(part 1 of 2)
# Autodesk Inventor assembly: Drive Roller Assembly 3 (Lexan)
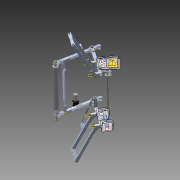
[picture p0: Inventor's stored thumbnail of the model, 180x180]
Saved by Autodesk Inventor 2014 (Build 180170000, 170)
## iProperties
Created: 2014-01-12
Part Number: Drive Roller Assembly 3 (Lexan)
Document SubType Name: Assembly
Designer: Michael
Mass: 8436.07 g
Surface Area: 19089.5 cm^2
Volume: 2323.39 cm^3
Density: 3.63094 g/cm^3
Author: Michael
## Documents named in this file (43)
- C:\Users\Michael\Documents\GitHub\2014buildCAD\Duluth Collector\Drive Roller Assembly 3 (Lexan).iam
- C:\Users\Michael\Documents\GitHub\2014buildCAD\Collector\Roller End Cap Drive (3-D Printed).ipt
- C:\Users\Michael\Documents\GitHub\2014buildCAD\Collector\VersaPlanetary (Fixed).iam
- C:\Users\Michael\Documents\GitHub\2014buildCAD\New Collector\Polycarbonate Roller 2 OD 1-16 Thick (8585K64).ipt
- C:\Users\Michael\Documents\GitHub\2014buildCAD\New Collector\Hex Bearing 1-2 in (FR8ZZ-Hex, am-0279).ipt
- C:\Users\Michael\Documents\GitHub\2014buildCAD\New Collector\Hex Shaft Collar 1-2 in (7552K500).ipt
- C:\Users\Michael\Documents\GitHub\2014buildCAD\New Collector\Roller End Cap Drive (3-D Printed).ipt
- C:\Users\Michael\Documents\GitHub\2014buildCAD\New Collector\Vex Pro End Bearing Mount.ipt
- C:\Users\Michael\Documents\GitHub\2014buildCAD\New Collector\Vex Pro 1x1 rectangular tubing 14 in length.ipt
- C:\Users\Michael\Documents\GitHub\2014buildCAD\New Collector\Hex Shaft Aluminum 1-2 in (am-2291).ipt
- C:\Users\Michael\Documents\GitHub\2014buildCAD\New Collector\Timing Pulley (HTD 5mm) - 18T 9mm Double Flange, 1-2 in Hex (VexPro).ipt
- C:\Users\Michael\Documents\GitHub\2014buildCAD\New Collector\Vex Pro 90 degree gusset.ipt
- C:\Users\Michael\Documents\GitHub\2014buildCAD\New Collector\Vex Pro 1x1 rectangular tubing 2 in length.ipt
- C:\Users\Michael\Documents\GitHub\2014buildCAD\New Collector\Hex Shaft 3-8 in (am-0855).ipt
- C:\Users\Michael\Documents\GitHub\2014buildCAD\New Collector\Hex Shaft Collar 3-8 in (7552K300).ipt
- C:\Users\Michael\Documents\GitHub\2014buildCAD\New Collector\Hex Shaft 1-2 in (am-0856).ipt
- C:\Users\Michael\Documents\GitHub\2014buildCAD\New Collector\Vex Pro 1x1 rectangular tubing 4 in length.ipt
- C:\Users\Michael\Documents\GitHub\2014buildCAD\New Collector\Pneumatic Piston Front Flange (Lt Custom).ipt
- C:\Users\Michael\Documents\GitHub\2014buildCAD\New Collector\Pneumatic Piston Front Flange (Rt Custom).ipt
- C:\Users\Michael\Documents\GitHub\2014buildCAD\New Collector\Pneumatic Piston Back Flange (Rt Custom).ipt
- C:\Users\Michael\Documents\GitHub\2014buildCAD\New Collector\Vex Pro 1x1 rectangular tubing 14 in length (roller).ipt
- C:\Users\Michael\Documents\GitHub\2014buildCAD\New Collector\Pneumatic Piston Back Flange (Right Custom).ipt
- C:\Users\Michael\Documents\GitHub\2014buildCAD\New Collector\Hex Shaft 1-2 in 5 in long (am-0856).ipt
- C:\Users\Michael\Documents\GitHub\2014buildCAD\New Collector\Vex Pro End Bearing Mount (Bolt).ipt
- C:\Users\Michael\Documents\GitHub\2014buildCAD\New Collector\Bracket.ipt
- C:\Users\Michael\Documents\GitHub\2014buildCAD\New Collector\Shaft Collar 3-16 in ID (6435K510).ipt
- C:\Users\Michael\Documents\GitHub\2014buildCAD\New Collector\Standoff #8 (91125A459).ipt
- C:\Users\Michael\Documents\GitHub\2014buildCAD\New Collector\Vex Pro 1x1 rectangular tubing 21.375 in length.ipt
- C:\Users\Michael\Documents\GitHub\2014buildCAD\New Collector\Roller Crossbar Gusset (Custom).ipt
- C:\Users\Michael\Documents\GitHub\2014buildCAD\New Collector\Vex Pro 1x1 rectangular tubing 2 in length (Flange Support).ipt
- C:\Users\Michael\Documents\GitHub\2014buildCAD\New Collector\Vex Pro 90 degree gusset (1-8 in).ipt
- C:\Users\Michael\Documents\GitHub\2014buildCAD\New Collector\Timing Pulley (HTD 5mm) - 18T 15mm 1-2 in Hex.ipt
- C:\Users\Michael\Documents\GitHub\2014buildCAD\New Collector\Hex Spacer.ipt
- C:\Users\Michael\Documents\GitHub\2014buildCAD\New Collector\Side Mount Custom.ipt
- C:\Users\Michael\Documents\GitHub\2014buildCAD\New Collector\Clamp Piston ( 1 in stroke twice, 9-16 bore).iam
- C:\Users\Michael\Documents\GitHub\2014buildCAD\New Collector\Hex Spacer 1-2 .ipt
- C:\Users\Michael\Documents\GitHub\2014buildCAD\New Collector\Lexan flexible Arm Mount.ipt
- C:\Users\Michael\Documents\GitHub\2014buildCAD\New Collector\Hex Shaft Connector (Lexan).ipt
- C:\Users\Michael\Documents\GitHub\2014buildCAD\New Collector\Clamp with Piston Assembly (new).iam
- C:\Users\Michael\Documents\GitHub\2014buildCAD\Duluth Collector\Vex Pro T gusset - OUT OF STOCK 1192014.ipt
- C:\Users\Michael\Documents\GitHub\2014buildCAD\Duluth Collector\Vex Pro 1x1 rectangular tubing 2 in length (no hex).ipt
- C:\Users\Michael\Documents\GitHub\2014buildCAD\Duluth Collector\Torsion Spring 10 in-lb (9271K621).ipt
- C:\Users\Michael\Documents\GitHub\2014buildCAD\Duluth Collector\Bearing Mount Spacer 1-8 in.ipt
## Components (143 placed, 41 different names)
1. Roller End Cap Drive (3-D Printed):2 — Mate:154, Mate:155, Mate:1112, Flush:30, Mate:1114, Mate:1115
2. VersaPlanetary (Fixed):1 [sub-assembly] — Mate:990, Mate:991, Mate:992, Mate:1076, Mate:1077, Mate:1079, Mate:1080, Mate:1082, Mate:1083
3. Hex Bearing 1-2 in (FR8ZZ-Hex, am-0279):3 — Mate:128, Mate:129, Mate:134, Mate:1113
4. Roller End Cap Drive (3-D Printed):5 — Mate:1108, Mate:1109, Mate:1110
5. Hex Shaft Aluminum 1-2 in (am-2291):1 — Mate:132, Mate:134, Mate:154, Mate:155, Mate:172, Mate:173, Mate:179, Mate:180, Mate:467, Mate:468, Mate:1065, Mate:1066, Mate:1068, Mate:1069, Mate:1072, Mate:1073, Flush:30
6. Vex Pro End Bearing Mount:4 — Mate:130, Mate:131, Mate:621, Mate:798, Mate:799, Mate:873
7. Vex Pro End Bearing Mount:5 — Mate:128, Mate:129, Mate:624, Mate:800, Mate:801, Mate:866, Mate:867, Mate:868, Mate:869, Mate:870, Mate:871, Mate:872
8. Hex Bearing 1-2 in (FR8ZZ-Hex, am-0279):4 — Mate:130, Mate:131, Mate:132, Mate:1067
9. Hex Bearing 1-2 in (FR8ZZ-Hex, am-0279):5 — Mate:178, Mate:758, Mate:759
10. Vex Pro End Bearing Mount:7 — Mate:631, Mate:804, Mate:805
11. Vex Pro End Bearing Mount:8 — Mate:629, Mate:802, Mate:803, Mate:874, Mate:875, Mate:876, Mate:877, Mate:878, Mate:879, Mate:880, Mate:881
12. Hex Bearing 1-2 in (FR8ZZ-Hex, am-0279):6 — Mate:172, Mate:173, Mate:470, Mate:471, Mate:1111
13. Hex Shaft Collar 1-2 in (7552K500):16 — Mate:178, Mate:179, Mate:180, Flush:13
14. Vex Pro 1x1 rectangular tubing 14 in length:5 — Mate:203, Mate:210, Mate:211, Mate:221, Mate:222, Mate:223, Flush:20, Mate:940, Mate:942, Mate:979, Mate:981, Flush:27, Mate:1084, Mate:1085, Mate:1140, Mate:1141, Mate:1146, Mate:1147, Mate:1148, Mate:1184, Mate:1185, Mate:1186, Mate:1190, Mate:1191, Mate:1192, Mate:1218, Mate:1219, Mate:1220, Mate:1224, Mate:1225, Mate:1226, Mate:1246, Mate:1247, Mate:1248, Mate:1250, Mate:1251, Mate:1252
15. Vex Pro 1x1 rectangular tubing 14 in length:6 — Mate:258, Mate:259, Mate:260, Mate:263, Mate:320, Mate:321, Flush:20, Mate:935, Mate:936, Mate:938, Mate:977, Flush:26, Mate:1092, Mate:1117, Mate:1129, Mate:1130, Mate:1131, Mate:1132, Mate:1230, Mate:1231, Mate:1232, Mate:1236, Mate:1237, Mate:1238, Mate:1254, Mate:1255, Mate:1256, Mate:1260, Mate:1261, Mate:1262
16. Vex Pro 90 degree gusset:8 — Mate:203, Mate:210, Mate:211, Mate:212, Mate:213, Mate:214
17. Vex Pro 1x1 rectangular tubing 2 in length:1 — Mate:212, Mate:213, Mate:214, Flush:25, Mate:941, Mate:961, Mate:962, Mate:964, Mate:965, Flush:37
18. Vex Pro 90 degree gusset:10 — Mate:221, Mate:222, Mate:223
19. Vex Pro 1x1 rectangular tubing 2 in length:2 — Mate:224, Mate:225, Mate:967, Mate:968, Mate:970, Mate:971, Mate:1086, Flush:38
20. Hex Shaft 3-8 in (am-0855):1 — Mate:224, Mate:225, Mate:228, Mate:229, Mate:231, Mate:232, Mate:919, Mate:920, Mate:922, Mate:923, Mate:963, Mate:966, Mate:969, Mate:972, Flush:32, Flush:33
21. Hex Shaft Collar 3-8 in (7552K300):1 — Mate:228, Mate:229, Mate:1163, Mate:1167, Mate:1242, Mate:1243, Flush:41
22. Hex Shaft Collar 3-8 in (7552K300):2 — Mate:231, Mate:232, Mate:1164, Flush:32
23. Vex Pro 90 degree gusset:12 — Mate:263, Mate:320, Mate:321
24. Vex Pro 1x1 rectangular tubing 2 in length:3 — Flush:25, Mate:949, Mate:950, Mate:952, Mate:953, Flush:40
25. Vex Pro 90 degree gusset:13 — Mate:258, Mate:259, Mate:260
26. Vex Pro 1x1 rectangular tubing 2 in length:4 — Mate:955, Mate:956, Mate:958, Mate:959, Mate:1090, Mate:1091
27. Hex Shaft 3-8 in (am-0855):2 — Mate:915, Mate:917, Mate:925, Mate:926, Mate:951, Mate:954, Mate:957, Mate:960, Flush:34
28. Hex Shaft Collar 3-8 in (7552K300):3 — Mate:1170, Mate:1183, Mate:1244, Mate:1245, Flush:42
29. Hex Shaft Collar 3-8 in (7552K300):4 — Mate:1159, Flush:34
30. Hex Shaft Collar 1-2 in (7552K500):18 — Mate:1150
31. Hex Shaft Collar 1-2 in (7552K500):19 — Mate:1149
32. Hex Shaft Collar 1-2 in (7552K500):20 — Mate:706, Mate:707, Mate:945
33. Hex Shaft Collar 1-2 in (7552K500):21 — Mate:704, Mate:705, Flush:22, Mate:1136
34. Hex Shaft Collar 1-2 in (7552K500):22 — Mate:467, Mate:468, Mate:1112, Mate:1113
35. Hex Shaft Aluminum 1-2 in (am-2291):2 — Mate:470, Mate:471, Flush:13, Mate:633, Mate:634, Mate:758, Mate:759, Mate:1108, Mate:1109
36. Vex Pro 1x1 rectangular tubing 4 in length:1 — Mate:683, Mate:684, Mate:685, Mate:1249, Mate:1253, Mate:1258, Mate:1265
37. Vex Pro 1x1 rectangular tubing 4 in length:2 — Mate:694, Mate:699, Mate:700, Mate:1257, Mate:1259, Mate:1263, Mate:1264
38. Hex Bearing 1-2 in (FR8ZZ-Hex, am-0279):7 — Flush:15, Mate:560, Mate:561, Flush:23, Mate:754, Mate:755, Mate:830
39. Hex Shaft 1-2 in (am-0856):4 — Mate:560, Mate:561, Mate:562, Mate:563, Flush:23, Mate:774, Mate:829, Mate:831, Mate:833, Mate:834, Mate:1040, Mate:1043
40. Hex Bearing 1-2 in (FR8ZZ-Hex, am-0279):8 — Flush:15, Mate:746, Mate:747, Mate:774, Mate:832
41. Vex Pro 1x1 rectangular tubing 14 in length (roller):1 — Mate:562, Mate:563, Mate:621, Mate:624, Mate:790, Mate:791, Mate:793, Mate:798, Mate:799, Mate:800, Mate:801, Mate:862, Mate:863, Mate:864, Mate:912, Mate:988, Mate:989, Mate:1038, Mate:1039, Mate:1041, Mate:1042, Flush:26, Mate:1050, Mate:1195, Mate:1196, Mate:1214, Mate:1215, Mate:1216
42. Hex Bearing 1-2 in (FR8ZZ-Hex, am-0279):9 — Flush:19, Mate:752, Mate:753, Mate:854
43. Hex Shaft 1-2 in (am-0856):5 — Flush:19, Mate:775, Mate:836, Mate:843, Mate:852, Mate:853, Mate:1046, Mate:1049
44. Hex Bearing 1-2 in (FR8ZZ-Hex, am-0279):10 — Mate:738, Mate:739, Mate:775, Mate:835
45. Vex Pro 1x1 rectangular tubing 14 in length (roller):2 — Mate:629, Mate:631, Mate:802, Mate:803, Mate:804, Mate:805, Mate:806, Mate:807, Mate:808, Mate:809, Mate:810, Mate:811, Mate:892, Mate:1044, Mate:1045, Mate:1047, Mate:1048, Flush:27, Mate:1197, Mate:1198, Mate:1211, Mate:1212
46. Hex Shaft Collar 1-2 in (7552K500):23 — Mate:633, Mate:634, Mate:1110, Mate:1111
47. Pneumatic Piston Front Flange (Rt Custom):2 — Mate:932, Mate:933, Mate:934, Mate:1155, Mate:1156, Mate:1157
48. Pneumatic Piston Front Flange (Lt Custom):1 — Mate:929, Mate:930, Mate:931, Mate:1160, Mate:1161, Mate:1162
49. Pneumatic Piston Back Flange (Rt Custom):1 — Mate:683, Mate:684, Mate:685, Mate:1028, Mate:1029, Mate:1030
50. Pneumatic Piston Back Flange (Right Custom):1 — Mate:694, Mate:699, Mate:700, Mate:1024, Mate:1025, Mate:1026
51. Hex Shaft 1-2 in 5 in long (am-0856):1 — Mate:704, Mate:705, Mate:706, Mate:707, Flush:22, Mate:714, Mate:715, Mate:946, Mate:947, Mate:1032, Mate:1033, Mate:1133, Mate:1135
52. Hex Shaft Collar 1-2 in (7552K500):24 — Mate:714, Mate:715, Mate:948
53. Vex Pro End Bearing Mount (Bolt):1 — Mate:738, Mate:739, Mate:979, Mate:1221, Mate:1222, Mate:1223
54. Vex Pro End Bearing Mount (Bolt):2 — Mate:752, Mate:753, Mate:981, Mate:1227, Mate:1228, Mate:1229
55. Vex Pro End Bearing Mount (Bolt):3 — Mate:746, Mate:747, Mate:1233, Mate:1234, Mate:1235
56. Vex Pro End Bearing Mount (Bolt):4 — Mate:754, Mate:755, Mate:977, Mate:1239, Mate:1240, Mate:1241
57. Bracket:1 — Mate:790, Mate:791, Mate:793, Mate:860
58. Bracket:2 — Mate:806, Mate:807, Mate:808, Mate:856
59. Bracket:3 — Mate:809, Mate:810, Mate:811, Mate:858
60. Hex Shaft Collar 1-2 in (7552K500):25 — Mate:829, Mate:830, Mate:831
61. Hex Shaft Collar 1-2 in (7552K500):26 — Mate:832, Mate:833, Mate:834
62. Hex Shaft Collar 1-2 in (7552K500):27 — Mate:835, Mate:836, Mate:843
63. Hex Shaft Collar 1-2 in (7552K500):29 — Mate:852, Mate:853, Mate:854
64. Shaft Collar 3-16 in ID (6435K510):1 — Mate:858
65. Shaft Collar 3-16 in ID (6435K510):2 — Mate:856
66. Shaft Collar 3-16 in ID (6435K510):3 — Mate:860
67. Shaft Collar 3-16 in ID (6435K510):4 — Mate:865
68. Bracket:4 — Mate:862, Mate:863, Mate:864, Mate:865
69. Standoff #8 (91125A459):1 — Mate:866, Mate:867
70. Standoff #8 (91125A459):2 — Mate:868, Mate:869
71. Standoff #8 (91125A459):3 — Mate:870, Mate:871
72. Standoff #8 (91125A459):4 — Mate:872, Mate:873
73. Standoff #8 (91125A459):5 — Mate:874, Mate:875
74. Standoff #8 (91125A459):6 — Mate:876, Mate:877
75. Standoff #8 (91125A459):7 — Mate:878, Mate:879
76. Standoff #8 (91125A459):8 — Mate:880, Mate:881
77. Vex Pro 1x1 rectangular tubing 21.375 in length:1 — Mate:894, Mate:1199, Mate:1213
78. Roller Crossbar Gusset (Custom):4 — Mate:892, Mate:894, Mate:1197, Mate:1198, Mate:1199
79. Roller Crossbar Gusset (Custom):5 — Mate:912, Mate:1195, Mate:1196
80. Hex Shaft Collar 3-8 in (7552K300):5 — Mate:915, Mate:917, Mate:1206
81. Hex Shaft Collar 3-8 in (7552K300):6 — Mate:919, Mate:920, Mate:1205
82. Hex Shaft Collar 3-8 in (7552K300):7 — Mate:922, Mate:923, Mate:1166
83. Hex Shaft Collar 3-8 in (7552K300):8 — Mate:925, Mate:926, Mate:1168
84. Vex Pro 1x1 rectangular tubing 2 in length (Flange Support):1 — Mate:929, Mate:930, Mate:931
85. Vex Pro 1x1 rectangular tubing 2 in length (Flange Support):2 — Mate:932, Mate:933, Mate:934
86. Vex Pro 90 degree gusset (1-8 in):1 — Mate:935, Mate:936, Mate:938
87. Vex Pro 90 degree gusset (1-8 in):2 — Mate:940, Mate:941, Mate:942
88. Timing Pulley (HTD 5mm) - 18T 15mm 1-2 in Hex:1 — Mate:945, Mate:946, Mate:947, Mate:948
89. Hex Spacer:1 — Mate:949, Mate:950, Mate:951
90. Hex Spacer:2 — Mate:952, Mate:953, Mate:954
91. Hex Spacer:3 — Mate:955, Mate:956, Mate:957
92. Hex Spacer:4 — Mate:958, Mate:959, Mate:960
93. Hex Spacer:5 — Mate:961, Mate:962, Mate:963
94. Hex Spacer:6 — Mate:964, Mate:965, Mate:966
95. Hex Spacer:7 — Mate:967, Mate:968, Mate:969, Flush:33
96. Hex Spacer:8 — Mate:970, Mate:971, Mate:972
97. Side Mount Custom:1 — Mate:988, Mate:989, Mate:990, Mate:991, Mate:992, Mate:1050
98. Clamp Piston ( 1 in stroke twice, 9-16 bore):1 [sub-assembly] — Mate:1024, Mate:1025, Mate:1026
99. Clamp Piston ( 1 in stroke twice, 9-16 bore):2 [sub-assembly] — Mate:1028, Mate:1029, Mate:1030
100. Hex Shaft Collar 1-2 in (7552K500):30 — Mate:1032, Mate:1033, Mate:1134
101. Hex Spacer 1-2 :1 — Mate:1038, Mate:1039, Mate:1040
102. Hex Spacer 1-2 :2 — Mate:1041, Mate:1042, Mate:1043
103. Hex Spacer 1-2 :3 — Mate:1044, Mate:1045, Mate:1046
104. Hex Spacer 1-2 :4 — Mate:1047, Mate:1048, Mate:1049
105. Hex Shaft Collar 1-2 in (7552K500):31 — Mate:1065, Mate:1066, Mate:1067, Mate:1070
106. Timing Pulley (HTD 5mm) - 18T 9mm Double Flange, 1-2 in Hex (VexPro):5 — Mate:1068, Mate:1069, Mate:1070, Mate:1071
107. Hex Shaft Collar 1-2 in (7552K500):32 — Mate:1071, Mate:1072, Mate:1073, Flush:29
108. Hex Shaft Collar 1-2 in (7552K500):33 — Mate:1081, Mate:1082, Mate:1083
109. Timing Pulley (HTD 5mm) - 18T 9mm Double Flange, 1-2 in Hex (VexPro):6 — Mate:1078, Mate:1079, Mate:1080, Mate:1081
110. Hex Shaft Collar 1-2 in (7552K500):34 — Mate:1076, Flush:29, Mate:1077, Mate:1078
111. Vex Pro 90 degree gusset (1-8 in):3 — Mate:1084, Mate:1085, Mate:1086
112. Vex Pro 90 degree gusset (1-8 in):4 — Mate:1090, Mate:1091, Mate:1092
113. Polycarbonate Roller 2 OD 1-16 Thick (8585K64):1 — Mate:1114, Mate:1115
114. Lexan flexible Arm Mount:1 — Mate:1117, Mate:1126, Mate:1127, Mate:1128, Mate:1129, Mate:1130, Mate:1153
115. Lexan flexible Arm Mount:2 — Mate:1123, Mate:1124, Mate:1125, Mate:1131, Mate:1132, Mate:1153
116. Hex Shaft Connector (Lexan):1 — Mate:1123, Mate:1124, Mate:1125, Mate:1133, Mate:1134
117. Hex Shaft Connector (Lexan):2 — Mate:1126, Mate:1127, Mate:1128, Mate:1135, Mate:1136
118. Lexan flexible Arm Mount:3 — Mate:1140, Mate:1141, Mate:1154
119. Hex Shaft Connector (Lexan):3 — Mate:1150
120. Lexan flexible Arm Mount:4 — Mate:1146, Mate:1147, Mate:1148, Mate:1154
121. Hex Shaft Connector (Lexan):4 — Mate:1149
122. Clamp with Piston Assembly (new):1 [sub-assembly] — Mate:1155, Mate:1156, Mate:1157, Mate:1159, Mate:1168, Mate:1170, Mate:1183, Mate:1206, Mate:1207, Mate:1208
123. Clamp with Piston Assembly (new):2 [sub-assembly] — Mate:1160, Mate:1161, Mate:1162, Mate:1163, Mate:1164, Mate:1166, Mate:1167, Mate:1203, Mate:1204, Mate:1205
124. Vex Pro 1x1 rectangular tubing 4 in length:3 — Mate:1187, Flush:35, Mate:1194
125. Vex Pro T gusset - OUT OF STOCK 1192014:1 — Mate:1184, Mate:1185, Mate:1186, Mate:1187, Flush:35, Mate:1188, Mate:1189, Flush:36
126. Vex Pro 1x1 rectangular tubing 2 in length (no hex):1 — Mate:1188, Mate:1189, Flush:36, Mate:1193
127. Vex Pro T gusset - OUT OF STOCK 1192014:2 — Mate:1190, Mate:1191, Mate:1192, Mate:1193, Mate:1194
128. Torsion Spring 10 in-lb (9271K621):1 — Mate:1203, Flush:37
129. Torsion Spring 10 in-lb (9271K621):2 — Mate:1204, Flush:38
130. Torsion Spring 10 in-lb (9271K621):3 — Mate:1207
131. Torsion Spring 10 in-lb (9271K621):4 — Mate:1208, Flush:40
132. Roller Crossbar Gusset (Custom):6 — Mate:1211, Mate:1212, Mate:1213
133. Roller Crossbar Gusset (Custom):7 — Mate:1214, Mate:1215, Mate:1216
134. Bearing Mount Spacer 1-8 in:1 — Mate:1218, Mate:1219, Mate:1220, Mate:1221, Mate:1222, Mate:1223
135. Bearing Mount Spacer 1-8 in:2 — Mate:1224, Mate:1225, Mate:1226, Mate:1227, Mate:1228, Mate:1229
136. Bearing Mount Spacer 1-8 in:3 — Mate:1230, Mate:1231, Mate:1232, Mate:1233, Mate:1234, Mate:1235
137. Bearing Mount Spacer 1-8 in:5 — Mate:1236, Mate:1237, Mate:1238, Mate:1239, Mate:1240, Mate:1241
138. Hex Shaft 3-8 in (am-0855):3 — Mate:1242, Mate:1243, Flush:41
139. Hex Shaft 3-8 in (am-0855):4 — Mate:1244, Mate:1245, Flush:42
140. Vex Pro T gusset - OUT OF STOCK 1192014:3 — Mate:1246, Mate:1247, Mate:1248, Mate:1249, Mate:1258, Mate:1265
141. Vex Pro T gusset - OUT OF STOCK 1192014:4 — Mate:1250, Mate:1251, Mate:1252, Mate:1253
142. Vex Pro T gusset - OUT OF STOCK 1192014:5 — Mate:1254, Mate:1255, Mate:1256, Mate:1257, Mate:1259
143. Vex Pro T gusset - OUT OF STOCK 1192014:6 — Mate:1260, Mate:1261, Mate:1262, Mate:1263, Mate:1264
## Relationships (400: Mate 378, Flush 22)
- Mate:128: Hex Bearing 1-2 in (FR8ZZ-Hex, am-0279):3 ↔ Vex Pro End Bearing Mount:5
- Mate:129: Hex Bearing 1-2 in (FR8ZZ-Hex, am-0279):3 ↔ Vex Pro End Bearing Mount:5
- Mate:130: Vex Pro End Bearing Mount:4 ↔ Hex Bearing 1-2 in (FR8ZZ-Hex, am-0279):4
- Mate:131: Vex Pro End Bearing Mount:4 ↔ Hex Bearing 1-2 in (FR8ZZ-Hex, am-0279):4
- Mate:132: Hex Shaft Aluminum 1-2 in (am-2291):1 ↔ Hex Bearing 1-2 in (FR8ZZ-Hex, am-0279):4
- Mate:134: Hex Bearing 1-2 in (FR8ZZ-Hex, am-0279):3 ↔ Hex Shaft Aluminum 1-2 in (am-2291):1
- Mate:154: Roller End Cap Drive (3-D Printed):2 ↔ Hex Shaft Aluminum 1-2 in (am-2291):1
- Mate:155: Roller End Cap Drive (3-D Printed):2 ↔ Hex Shaft Aluminum 1-2 in (am-2291):1
- [Mate]: Hex Bearing 1-2 in (FR8ZZ-Hex, am-0279):5 ↔ Vex Pro End Bearing Mount:8
- [Mate]: Hex Bearing 1-2 in (FR8ZZ-Hex, am-0279):5 ↔ Vex Pro End Bearing Mount:8
- [Mate]: Vex Pro End Bearing Mount:7 ↔ Hex Bearing 1-2 in (FR8ZZ-Hex, am-0279):6
- [Mate]: Vex Pro End Bearing Mount:7 ↔ Hex Bearing 1-2 in (FR8ZZ-Hex, am-0279):6
- Mate:172: Hex Shaft Aluminum 1-2 in (am-2291):1 ↔ Hex Bearing 1-2 in (FR8ZZ-Hex, am-0279):6
- Mate:173: Hex Shaft Aluminum 1-2 in (am-2291):1 ↔ Hex Bearing 1-2 in (FR8ZZ-Hex, am-0279):6
- Mate:178: Hex Bearing 1-2 in (FR8ZZ-Hex, am-0279):5 ↔ Hex Shaft Collar 1-2 in (7552K500):16
- Mate:179: Hex Shaft Aluminum 1-2 in (am-2291):1 ↔ Hex Shaft Collar 1-2 in (7552K500):16
- Mate:180: Hex Shaft Aluminum 1-2 in (am-2291):1 ↔ Hex Shaft Collar 1-2 in (7552K500):16
- Mate:203: Vex Pro 1x1 rectangular tubing 14 in length:5 ↔ Vex Pro 90 degree gusset:8
- Mate:210: Vex Pro 1x1 rectangular tubing 14 in length:5 ↔ Vex Pro 90 degree gusset:8
- Mate:211: Vex Pro 1x1 rectangular tubing 14 in length:5 ↔ Vex Pro 90 degree gusset:8
- Mate:212: Vex Pro 90 degree gusset:8 ↔ Vex Pro 1x1 rectangular tubing 2 in length:1
- Mate:213: Vex Pro 90 degree gusset:8 ↔ Vex Pro 1x1 rectangular tubing 2 in length:1
- Mate:214: Vex Pro 90 degree gusset:8 ↔ Vex Pro 1x1 rectangular tubing 2 in length:1
- [Mate]: Vex Pro 90 degree gusset:10 ↔ Vex Pro 1x1 rectangular tubing 2 in length:2
- [Mate]: Vex Pro 90 degree gusset:10 ↔ Vex Pro 1x1 rectangular tubing 2 in length:2
- [Mate]: Vex Pro 90 degree gusset:10 ↔ Vex Pro 1x1 rectangular tubing 2 in length:2
- Mate:221: Vex Pro 1x1 rectangular tubing 14 in length:5 ↔ Vex Pro 90 degree gusset:10
- Mate:222: Vex Pro 1x1 rectangular tubing 14 in length:5 ↔ Vex Pro 90 degree gusset:10
- Mate:223: Vex Pro 1x1 rectangular tubing 14 in length:5 ↔ Vex Pro 90 degree gusset:10
- Mate:224: Vex Pro 1x1 rectangular tubing 2 in length:2 ↔ Hex Shaft 3-8 in (am-0855):1
- Mate:225: Vex Pro 1x1 rectangular tubing 2 in length:2 ↔ Hex Shaft 3-8 in (am-0855):1
- Mate:228: Hex Shaft 3-8 in (am-0855):1 ↔ Hex Shaft Collar 3-8 in (7552K300):1
- Mate:229: Hex Shaft 3-8 in (am-0855):1 ↔ Hex Shaft Collar 3-8 in (7552K300):1
- Mate:231: Hex Shaft 3-8 in (am-0855):1 ↔ Hex Shaft Collar 3-8 in (7552K300):2
- Mate:232: Hex Shaft 3-8 in (am-0855):1 ↔ Hex Shaft Collar 3-8 in (7552K300):2
- [Mate]: Vex Pro 90 degree gusset:12 ↔ Vex Pro 1x1 rectangular tubing 2 in length:3
- [Mate]: Vex Pro 90 degree gusset:13 ↔ Vex Pro 1x1 rectangular tubing 2 in length:4
- [Mate]: Vex Pro 90 degree gusset:13 ↔ Vex Pro 1x1 rectangular tubing 2 in length:4
- [Mate]: Vex Pro 90 degree gusset:13 ↔ Vex Pro 1x1 rectangular tubing 2 in length:4
- [Mate]: Vex Pro 1x1 rectangular tubing 2 in length:4 ↔ Hex Shaft 3-8 in (am-0855):2
- [Mate]: Vex Pro 1x1 rectangular tubing 2 in length:4 ↔ Hex Shaft 3-8 in (am-0855):2
- [Mate]: Hex Shaft 3-8 in (am-0855):2 ↔ Hex Shaft Collar 3-8 in (7552K300):3
- [Mate]: Hex Shaft 3-8 in (am-0855):2 ↔ Hex Shaft Collar 3-8 in (7552K300):3
- [Mate]: Hex Shaft 3-8 in (am-0855):2 ↔ Hex Shaft Collar 3-8 in (7552K300):4
- [Mate]: Hex Shaft 3-8 in (am-0855):2 ↔ Hex Shaft Collar 3-8 in (7552K300):4
- Mate:258: Vex Pro 1x1 rectangular tubing 14 in length:6 ↔ Vex Pro 90 degree gusset:13
- Mate:259: Vex Pro 1x1 rectangular tubing 14 in length:6 ↔ Vex Pro 90 degree gusset:13
- Mate:260: Vex Pro 1x1 rectangular tubing 14 in length:6 ↔ Vex Pro 90 degree gusset:13
- Mate:263: Vex Pro 1x1 rectangular tubing 14 in length:6 ↔ Vex Pro 90 degree gusset:12
- Mate:320: Vex Pro 1x1 rectangular tubing 14 in length:6 ↔ Vex Pro 90 degree gusset:12
- Mate:321: Vex Pro 1x1 rectangular tubing 14 in length:6 ↔ Vex Pro 90 degree gusset:12
- Mate:467: Hex Shaft Aluminum 1-2 in (am-2291):1 ↔ Hex Shaft Collar 1-2 in (7552K500):22
- Mate:468: Hex Shaft Aluminum 1-2 in (am-2291):1 ↔ Hex Shaft Collar 1-2 in (7552K500):22
- Mate:470: Hex Bearing 1-2 in (FR8ZZ-Hex, am-0279):6 ↔ Hex Shaft Aluminum 1-2 in (am-2291):2
- Mate:471: Hex Bearing 1-2 in (FR8ZZ-Hex, am-0279):6 ↔ Hex Shaft Aluminum 1-2 in (am-2291):2
- Flush:13 (-3.175 mm): Hex Shaft Collar 1-2 in (7552K500):16 ↔ Hex Shaft Aluminum 1-2 in (am-2291):2
- Flush:15: Hex Bearing 1-2 in (FR8ZZ-Hex, am-0279):7 ↔ Hex Bearing 1-2 in (FR8ZZ-Hex, am-0279):8
- Mate:560: Hex Bearing 1-2 in (FR8ZZ-Hex, am-0279):7 ↔ Hex Shaft 1-2 in (am-0856):4
- Mate:561: Hex Bearing 1-2 in (FR8ZZ-Hex, am-0279):7 ↔ Hex Shaft 1-2 in (am-0856):4
- Mate:562: Hex Shaft 1-2 in (am-0856):4 ↔ Vex Pro 1x1 rectangular tubing 14 in length (roller):1
- Mate:563: Hex Shaft 1-2 in (am-0856):4 ↔ Vex Pro 1x1 rectangular tubing 14 in length (roller):1
- [Flush]: Hex Bearing 1-2 in (FR8ZZ-Hex, am-0279):9 ↔ Hex Bearing 1-2 in (FR8ZZ-Hex, am-0279):10
- [Mate]: Hex Bearing 1-2 in (FR8ZZ-Hex, am-0279):9 ↔ Hex Shaft 1-2 in (am-0856):5
- [Mate]: Hex Bearing 1-2 in (FR8ZZ-Hex, am-0279):9 ↔ Hex Shaft 1-2 in (am-0856):5
- [Mate]: Hex Shaft 1-2 in (am-0856):5 ↔ Vex Pro 1x1 rectangular tubing 14 in length (roller):2
- [Mate]: Hex Shaft 1-2 in (am-0856):5 ↔ Vex Pro 1x1 rectangular tubing 14 in length (roller):2
- Flush:19 (15.0812 mm): Hex Bearing 1-2 in (FR8ZZ-Hex, am-0279):9 ↔ Hex Shaft 1-2 in (am-0856):5
- Mate:621: Vex Pro End Bearing Mount:4 ↔ Vex Pro 1x1 rectangular tubing 14 in length (roller):1
- Mate:624: Vex Pro End Bearing Mount:5 ↔ Vex Pro 1x1 rectangular tubing 14 in length (roller):1
- Mate:629: Vex Pro End Bearing Mount:8 ↔ Vex Pro 1x1 rectangular tubing 14 in length (roller):2
- Flush:20: Vex Pro 1x1 rectangular tubing 14 in length:5 ↔ Vex Pro 1x1 rectangular tubing 14 in length:6
- Mate:631: Vex Pro End Bearing Mount:7 ↔ Vex Pro 1x1 rectangular tubing 14 in length (roller):2
- Mate:633: Hex Shaft Aluminum 1-2 in (am-2291):2 ↔ Hex Shaft Collar 1-2 in (7552K500):23
- Mate:634: Hex Shaft Aluminum 1-2 in (am-2291):2 ↔ Hex Shaft Collar 1-2 in (7552K500):23
- Mate:683: Vex Pro 1x1 rectangular tubing 4 in length:1 ↔ Pneumatic Piston Back Flange (Rt Custom):1
- Mate:684: Vex Pro 1x1 rectangular tubing 4 in length:1 ↔ Pneumatic Piston Back Flange (Rt Custom):1
- Mate:685: Vex Pro 1x1 rectangular tubing 4 in length:1 ↔ Pneumatic Piston Back Flange (Rt Custom):1
- Mate:694: Vex Pro 1x1 rectangular tubing 4 in length:2 ↔ Pneumatic Piston Back Flange (Right Custom):1
- Mate:699: Vex Pro 1x1 rectangular tubing 4 in length:2 ↔ Pneumatic Piston Back Flange (Right Custom):1
- Mate:700: Vex Pro 1x1 rectangular tubing 4 in length:2 ↔ Pneumatic Piston Back Flange (Right Custom):1
- Mate:704: Hex Shaft Collar 1-2 in (7552K500):21 ↔ Hex Shaft 1-2 in 5 in long (am-0856):1
- Mate:705: Hex Shaft Collar 1-2 in (7552K500):21 ↔ Hex Shaft 1-2 in 5 in long (am-0856):1
- Mate:706: Hex Shaft Collar 1-2 in (7552K500):20 ↔ Hex Shaft 1-2 in 5 in long (am-0856):1
- Mate:707: Hex Shaft Collar 1-2 in (7552K500):20 ↔ Hex Shaft 1-2 in 5 in long (am-0856):1
- Flush:22 (-3.175 mm): Hex Shaft Collar 1-2 in (7552K500):21 ↔ Hex Shaft 1-2 in 5 in long (am-0856):1
- Mate:714: Hex Shaft 1-2 in 5 in long (am-0856):1 ↔ Hex Shaft Collar 1-2 in (7552K500):24
- Mate:715: Hex Shaft 1-2 in 5 in long (am-0856):1 ↔ Hex Shaft Collar 1-2 in (7552K500):24
- Mate:738: Hex Bearing 1-2 in (FR8ZZ-Hex, am-0279):10 ↔ Vex Pro End Bearing Mount (Bolt):1
- Mate:739: Hex Bearing 1-2 in (FR8ZZ-Hex, am-0279):10 ↔ Vex Pro End Bearing Mount (Bolt):1
- Flush:23 (-9.525 mm): Hex Bearing 1-2 in (FR8ZZ-Hex, am-0279):7 ↔ Hex Shaft 1-2 in (am-0856):4
- Mate:746: Hex Bearing 1-2 in (FR8ZZ-Hex, am-0279):8 ↔ Vex Pro End Bearing Mount (Bolt):3
- Mate:747: Hex Bearing 1-2 in (FR8ZZ-Hex, am-0279):8 ↔ Vex Pro End Bearing Mount (Bolt):3
- Mate:752: Hex Bearing 1-2 in (FR8ZZ-Hex, am-0279):9 ↔ Vex Pro End Bearing Mount (Bolt):2
- Mate:753: Hex Bearing 1-2 in (FR8ZZ-Hex, am-0279):9 ↔ Vex Pro End Bearing Mount (Bolt):2
- Mate:754: Hex Bearing 1-2 in (FR8ZZ-Hex, am-0279):7 ↔ Vex Pro End Bearing Mount (Bolt):4
- Mate:755: Hex Bearing 1-2 in (FR8ZZ-Hex, am-0279):7 ↔ Vex Pro End Bearing Mount (Bolt):4
- Mate:758: Hex Bearing 1-2 in (FR8ZZ-Hex, am-0279):5 ↔ Hex Shaft Aluminum 1-2 in (am-2291):2
- Mate:759: Hex Bearing 1-2 in (FR8ZZ-Hex, am-0279):5 ↔ Hex Shaft Aluminum 1-2 in (am-2291):2
- Mate:774: Hex Shaft 1-2 in (am-0856):4 ↔ Hex Bearing 1-2 in (FR8ZZ-Hex, am-0279):8
- Mate:775: Hex Shaft 1-2 in (am-0856):5 ↔ Hex Bearing 1-2 in (FR8ZZ-Hex, am-0279):10
- Mate:790: Vex Pro 1x1 rectangular tubing 14 in length (roller):1 ↔ Bracket:1
- Mate:791: Vex Pro 1x1 rectangular tubing 14 in length (roller):1 ↔ Bracket:1
- Mate:793: Vex Pro 1x1 rectangular tubing 14 in length (roller):1 ↔ Bracket:1
- Mate:798: Vex Pro End Bearing Mount:4 ↔ Vex Pro 1x1 rectangular tubing 14 in length (roller):1
- Mate:799: Vex Pro End Bearing Mount:4 ↔ Vex Pro 1x1 rectangular tubing 14 in length (roller):1
- Mate:800: Vex Pro End Bearing Mount:5 ↔ Vex Pro 1x1 rectangular tubing 14 in length (roller):1
- Mate:801: Vex Pro End Bearing Mount:5 ↔ Vex Pro 1x1 rectangular tubing 14 in length (roller):1
- Mate:802: Vex Pro End Bearing Mount:8 ↔ Vex Pro 1x1 rectangular tubing 14 in length (roller):2
- Mate:803: Vex Pro End Bearing Mount:8 ↔ Vex Pro 1x1 rectangular tubing 14 in length (roller):2
- Mate:804: Vex Pro End Bearing Mount:7 ↔ Vex Pro 1x1 rectangular tubing 14 in length (roller):2
- Mate:805: Vex Pro End Bearing Mount:7 ↔ Vex Pro 1x1 rectangular tubing 14 in length (roller):2
- Mate:806: Vex Pro 1x1 rectangular tubing 14 in length (roller):2 ↔ Bracket:2
- Mate:807: Vex Pro 1x1 rectangular tubing 14 in length (roller):2 ↔ Bracket:2
- Mate:808: Vex Pro 1x1 rectangular tubing 14 in length (roller):2 ↔ Bracket:2
- Mate:809: Vex Pro 1x1 rectangular tubing 14 in length (roller):2 ↔ Bracket:3
- Mate:810: Vex Pro 1x1 rectangular tubing 14 in length (roller):2 ↔ Bracket:3
- Mate:811: Vex Pro 1x1 rectangular tubing 14 in length (roller):2 ↔ Bracket:3
- Flush:25: Vex Pro 1x1 rectangular tubing 2 in length:1 ↔ Vex Pro 1x1 rectangular tubing 2 in length:3
- Mate:829: Hex Shaft 1-2 in (am-0856):4 ↔ Hex Shaft Collar 1-2 in (7552K500):25
- Mate:830: Hex Bearing 1-2 in (FR8ZZ-Hex, am-0279):7 ↔ Hex Shaft Collar 1-2 in (7552K500):25
- Mate:831: Hex Shaft 1-2 in (am-0856):4 ↔ Hex Shaft Collar 1-2 in (7552K500):25
- Mate:832: Hex Bearing 1-2 in (FR8ZZ-Hex, am-0279):8 ↔ Hex Shaft Collar 1-2 in (7552K500):26
- Mate:833: Hex Shaft 1-2 in (am-0856):4 ↔ Hex Shaft Collar 1-2 in (7552K500):26
- Mate:834: Hex Shaft 1-2 in (am-0856):4 ↔ Hex Shaft Collar 1-2 in (7552K500):26
- Mate:835: Hex Bearing 1-2 in (FR8ZZ-Hex, am-0279):10 ↔ Hex Shaft Collar 1-2 in (7552K500):27
- Mate:836: Hex Shaft 1-2 in (am-0856):5 ↔ Hex Shaft Collar 1-2 in (7552K500):27
- Mate:843: Hex Shaft 1-2 in (am-0856):5 ↔ Hex Shaft Collar 1-2 in (7552K500):27
- Mate:852: Hex Shaft 1-2 in (am-0856):5 ↔ Hex Shaft Collar 1-2 in (7552K500):29
- Mate:853: Hex Shaft 1-2 in (am-0856):5 ↔ Hex Shaft Collar 1-2 in (7552K500):29
- Mate:854: Hex Bearing 1-2 in (FR8ZZ-Hex, am-0279):9 ↔ Hex Shaft Collar 1-2 in (7552K500):29
- Mate:856: Bracket:2 ↔ Shaft Collar 3-16 in ID (6435K510):2
- Mate:858: Bracket:3 ↔ Shaft Collar 3-16 in ID (6435K510):1
- Mate:860: Bracket:1 ↔ Shaft Collar 3-16 in ID (6435K510):3
- Mate:862: Vex Pro 1x1 rectangular tubing 14 in length (roller):1 ↔ Bracket:4
- Mate:863: Vex Pro 1x1 rectangular tubing 14 in length (roller):1 ↔ Bracket:4
- Mate:864: Vex Pro 1x1 rectangular tubing 14 in length (roller):1 ↔ Bracket:4
- Mate:865: Shaft Collar 3-16 in ID (6435K510):4 ↔ Bracket:4
- Mate:866: Vex Pro End Bearing Mount:5 ↔ Standoff #8 (91125A459):1
- Mate:867: Vex Pro End Bearing Mount:5 ↔ Standoff #8 (91125A459):1
- Mate:868: Vex Pro End Bearing Mount:5 ↔ Standoff #8 (91125A459):2
- Mate:869: Vex Pro End Bearing Mount:5 ↔ Standoff #8 (91125A459):2
- Mate:870: Vex Pro End Bearing Mount:5 ↔ Standoff #8 (91125A459):3
- Mate:871: Vex Pro End Bearing Mount:5 ↔ Standoff #8 (91125A459):3
- Mate:872: Vex Pro End Bearing Mount:5 ↔ Standoff #8 (91125A459):4
- Mate:873: Vex Pro End Bearing Mount:4 ↔ Standoff #8 (91125A459):4
- Mate:874: Vex Pro End Bearing Mount:8 ↔ Standoff #8 (91125A459):5
- Mate:875: Vex Pro End Bearing Mount:8 ↔ Standoff #8 (91125A459):5
- Mate:876: Vex Pro End Bearing Mount:8 ↔ Standoff #8 (91125A459):6
- Mate:877: Vex Pro End Bearing Mount:8 ↔ Standoff #8 (91125A459):6
- Mate:878: Vex Pro End Bearing Mount:8 ↔ Standoff #8 (91125A459):7
- Mate:879: Vex Pro End Bearing Mount:8 ↔ Standoff #8 (91125A459):7
- Mate:880: Vex Pro End Bearing Mount:8 ↔ Standoff #8 (91125A459):8
- Mate:881: Vex Pro End Bearing Mount:8 ↔ Standoff #8 (91125A459):8
- Mate:892: Vex Pro 1x1 rectangular tubing 14 in length (roller):2 ↔ Roller Crossbar Gusset (Custom):4
- Mate:894: Vex Pro 1x1 rectangular tubing 21.375 in length:1 ↔ Roller Crossbar Gusset (Custom):4
- Mate:912: Vex Pro 1x1 rectangular tubing 14 in length (roller):1 ↔ Roller Crossbar Gusset (Custom):5
- Mate:915: Hex Shaft 3-8 in (am-0855):2 ↔ Hex Shaft Collar 3-8 in (7552K300):5
- Mate:917: Hex Shaft 3-8 in (am-0855):2 ↔ Hex Shaft Collar 3-8 in (7552K300):5
- Mate:919: Hex Shaft 3-8 in (am-0855):1 ↔ Hex Shaft Collar 3-8 in (7552K300):6
- Mate:920: Hex Shaft 3-8 in (am-0855):1 ↔ Hex Shaft Collar 3-8 in (7552K300):6
- Mate:922: Hex Shaft 3-8 in (am-0855):1 ↔ Hex Shaft Collar 3-8 in (7552K300):7
- Mate:923: Hex Shaft 3-8 in (am-0855):1 ↔ Hex Shaft Collar 3-8 in (7552K300):7
- Mate:925: Hex Shaft 3-8 in (am-0855):2 ↔ Hex Shaft Collar 3-8 in (7552K300):8
- Mate:926: Hex Shaft 3-8 in (am-0855):2 ↔ Hex Shaft Collar 3-8 in (7552K300):8
- Mate:929: Pneumatic Piston Front Flange (Lt Custom):1 ↔ Vex Pro 1x1 rectangular tubing 2 in length (Flange Support):1
- Mate:930: Pneumatic Piston Front Flange (Lt Custom):1 ↔ Vex Pro 1x1 rectangular tubing 2 in length (Flange Support):1
- Mate:931: Pneumatic Piston Front Flange (Lt Custom):1 ↔ Vex Pro 1x1 rectangular tubing 2 in length (Flange Support):1
- Mate:932: Pneumatic Piston Front Flange (Rt Custom):2 ↔ Vex Pro 1x1 rectangular tubing 2 in length (Flange Support):2
- Mate:933: Pneumatic Piston Front Flange (Rt Custom):2 ↔ Vex Pro 1x1 rectangular tubing 2 in length (Flange Support):2
- Mate:934: Pneumatic Piston Front Flange (Rt Custom):2 ↔ Vex Pro 1x1 rectangular tubing 2 in length (Flange Support):2
- Mate:935: Vex Pro 1x1 rectangular tubing 14 in length:6 ↔ Vex Pro 90 degree gusset (1-8 in):1
- Mate:936: Vex Pro 1x1 rectangular tubing 14 in length:6 ↔ Vex Pro 90 degree gusset (1-8 in):1
- Mate:938: Vex Pro 1x1 rectangular tubing 14 in length:6 ↔ Vex Pro 90 degree gusset (1-8 in):1
- Mate:940: Vex Pro 1x1 rectangular tubing 14 in length:5 ↔ Vex Pro 90 degree gusset (1-8 in):2
- Mate:941: Vex Pro 1x1 rectangular tubing 2 in length:1 ↔ Vex Pro 90 degree gusset (1-8 in):2
- Mate:942: Vex Pro 1x1 rectangular tubing 14 in length:5 ↔ Vex Pro 90 degree gusset (1-8 in):2
- Mate:945: Hex Shaft Collar 1-2 in (7552K500):20 ↔ Timing Pulley (HTD 5mm) - 18T 15mm 1-2 in Hex:1
- Mate:946: Hex Shaft 1-2 in 5 in long (am-0856):1 ↔ Timing Pulley (HTD 5mm) - 18T 15mm 1-2 in Hex:1
- Mate:947: Hex Shaft 1-2 in 5 in long (am-0856):1 ↔ Timing Pulley (HTD 5mm) - 18T 15mm 1-2 in Hex:1
- Mate:948: Hex Shaft Collar 1-2 in (7552K500):24 ↔ Timing Pulley (HTD 5mm) - 18T 15mm 1-2 in Hex:1
- Mate:949: Vex Pro 1x1 rectangular tubing 2 in length:3 ↔ Hex Spacer:1
- Mate:950: Vex Pro 1x1 rectangular tubing 2 in length:3 ↔ Hex Spacer:1
- Mate:951: Hex Shaft 3-8 in (am-0855):2 ↔ Hex Spacer:1
- Mate:952: Vex Pro 1x1 rectangular tubing 2 in length:3 ↔ Hex Spacer:2
- Mate:953: Vex Pro 1x1 rectangular tubing 2 in length:3 ↔ Hex Spacer:2
- Mate:954: Hex Shaft 3-8 in (am-0855):2 ↔ Hex Spacer:2
- Mate:955: Vex Pro 1x1 rectangular tubing 2 in length:4 ↔ Hex Spacer:3
- Mate:956: Vex Pro 1x1 rectangular tubing 2 in length:4 ↔ Hex Spacer:3
- Mate:957: Hex Shaft 3-8 in (am-0855):2 ↔ Hex Spacer:3
- Mate:958: Vex Pro 1x1 rectangular tubing 2 in length:4 ↔ Hex Spacer:4
- Mate:959: Vex Pro 1x1 rectangular tubing 2 in length:4 ↔ Hex Spacer:4
- Mate:960: Hex Shaft 3-8 in (am-0855):2 ↔ Hex Spacer:4
- Mate:961: Vex Pro 1x1 rectangular tubing 2 in length:1 ↔ Hex Spacer:5
- Mate:962: Vex Pro 1x1 rectangular tubing 2 in length:1 ↔ Hex Spacer:5
- Mate:963: Hex Shaft 3-8 in (am-0855):1 ↔ Hex Spacer:5
- Mate:964: Vex Pro 1x1 rectangular tubing 2 in length:1 ↔ Hex Spacer:6
- Mate:965: Vex Pro 1x1 rectangular tubing 2 in length:1 ↔ Hex Spacer:6
- Mate:966: Hex Shaft 3-8 in (am-0855):1 ↔ Hex Spacer:6
- Mate:967: Vex Pro 1x1 rectangular tubing 2 in length:2 ↔ Hex Spacer:7
- Mate:968: Vex Pro 1x1 rectangular tubing 2 in length:2 ↔ Hex Spacer:7
- Mate:969: Hex Shaft 3-8 in (am-0855):1 ↔ Hex Spacer:7
- Mate:970: Vex Pro 1x1 rectangular tubing 2 in length:2 ↔ Hex Spacer:8
- Mate:971: Vex Pro 1x1 rectangular tubing 2 in length:2 ↔ Hex Spacer:8
- Mate:972: Hex Shaft 3-8 in (am-0855):1 ↔ Hex Spacer:8
- Mate:977: Vex Pro 1x1 rectangular tubing 14 in length:6 ↔ Vex Pro End Bearing Mount (Bolt):4
- Mate:979: Vex Pro 1x1 rectangular tubing 14 in length:5 ↔ Vex Pro End Bearing Mount (Bolt):1
- Mate:981: Vex Pro 1x1 rectangular tubing 14 in length:5 ↔ Vex Pro End Bearing Mount (Bolt):2
- Mate:988: Vex Pro 1x1 rectangular tubing 14 in length (roller):1 ↔ Side Mount Custom:1
- Mate:989: Vex Pro 1x1 rectangular tubing 14 in length (roller):1 ↔ Side Mount Custom:1
- Mate:990: VersaPlanetary (Fixed):1 ↔ Side Mount Custom:1
- Mate:991: VersaPlanetary (Fixed):1 ↔ Side Mount Custom:1
- Mate:992: VersaPlanetary (Fixed):1 ↔ Side Mount Custom:1
- Mate:1024: Pneumatic Piston Back Flange (Right Custom):1 ↔ Clamp Piston ( 1 in stroke twice, 9-16 bore):1
- Mate:1025: Pneumatic Piston Back Flange (Right Custom):1 ↔ Clamp Piston ( 1 in stroke twice, 9-16 bore):1
- Mate:1026: Pneumatic Piston Back Flange (Right Custom):1 ↔ Clamp Piston ( 1 in stroke twice, 9-16 bore):1
- Mate:1028: Pneumatic Piston Back Flange (Rt Custom):1 ↔ Clamp Piston ( 1 in stroke twice, 9-16 bore):2
- Mate:1029: Pneumatic Piston Back Flange (Rt Custom):1 ↔ Clamp Piston ( 1 in stroke twice, 9-16 bore):2
- Mate:1030: Pneumatic Piston Back Flange (Rt Custom):1 ↔ Clamp Piston ( 1 in stroke twice, 9-16 bore):2
- Mate:1032: Hex Shaft 1-2 in 5 in long (am-0856):1 ↔ Hex Shaft Collar 1-2 in (7552K500):30
- Mate:1033: Hex Shaft 1-2 in 5 in long (am-0856):1 ↔ Hex Shaft Collar 1-2 in (7552K500):30
- Mate:1038: Vex Pro 1x1 rectangular tubing 14 in length (roller):1 ↔ Hex Spacer 1-2 :1
- Mate:1039: Vex Pro 1x1 rectangular tubing 14 in length (roller):1 ↔ Hex Spacer 1-2 :1
- Mate:1040: Hex Shaft 1-2 in (am-0856):4 ↔ Hex Spacer 1-2 :1
- Mate:1041: Vex Pro 1x1 rectangular tubing 14 in length (roller):1 ↔ Hex Spacer 1-2 :2
- Mate:1042: Vex Pro 1x1 rectangular tubing 14 in length (roller):1 ↔ Hex Spacer 1-2 :2
- Mate:1043: Hex Shaft 1-2 in (am-0856):4 ↔ Hex Spacer 1-2 :2
- Mate:1044: Vex Pro 1x1 rectangular tubing 14 in length (roller):2 ↔ Hex Spacer 1-2 :3
- Mate:1045: Vex Pro 1x1 rectangular tubing 14 in length (roller):2 ↔ Hex Spacer 1-2 :3
- Mate:1046: Hex Shaft 1-2 in (am-0856):5 ↔ Hex Spacer 1-2 :3
- Mate:1047: Vex Pro 1x1 rectangular tubing 14 in length (roller):2 ↔ Hex Spacer 1-2 :4
- Mate:1048: Vex Pro 1x1 rectangular tubing 14 in length (roller):2 ↔ Hex Spacer 1-2 :4
- Mate:1049: Hex Shaft 1-2 in (am-0856):5 ↔ Hex Spacer 1-2 :4
- Flush:26: Vex Pro 1x1 rectangular tubing 14 in length:6 ↔ Vex Pro 1x1 rectangular tubing 14 in length (roller):1
- Mate:1050: Vex Pro 1x1 rectangular tubing 14 in length (roller):1 ↔ Side Mount Custom:1
- Flush:27: Vex Pro 1x1 rectangular tubing 14 in length:5 ↔ Vex Pro 1x1 rectangular tubing 14 in length (roller):2
- Mate:1065: Hex Shaft Aluminum 1-2 in (am-2291):1 ↔ Hex Shaft Collar 1-2 in (7552K500):31
- Mate:1066: Hex Shaft Aluminum 1-2 in (am-2291):1 ↔ Hex Shaft Collar 1-2 in (7552K500):31
- Mate:1067: Hex Bearing 1-2 in (FR8ZZ-Hex, am-0279):4 ↔ Hex Shaft Collar 1-2 in (7552K500):31
- Mate:1068: Hex Shaft Aluminum 1-2 in (am-2291):1 ↔ Timing Pulley (HTD 5mm) - 18T 9mm Double Flange, 1-2 in Hex (VexPro):5
- Mate:1069: Hex Shaft Aluminum 1-2 in (am-2291):1 ↔ Timing Pulley (HTD 5mm) - 18T 9mm Double Flange, 1-2 in Hex (VexPro):5
- Mate:1070: Hex Shaft Collar 1-2 in (7552K500):31 ↔ Timing Pulley (HTD 5mm) - 18T 9mm Double Flange, 1-2 in Hex (VexPro):5
- Mate:1071: Timing Pulley (HTD 5mm) - 18T 9mm Double Flange, 1-2 in Hex (VexPro):5 ↔ Hex Shaft Collar 1-2 in (7552K500):32
- Mate:1072: Hex Shaft Aluminum 1-2 in (am-2291):1 ↔ Hex Shaft Collar 1-2 in (7552K500):32
- Mate:1073: Hex Shaft Aluminum 1-2 in (am-2291):1 ↔ Hex Shaft Collar 1-2 in (7552K500):32
- [Mate]: Hex Shaft Collar 1-2 in (7552K500):33 ↔ Timing Pulley (HTD 5mm) - 18T 9mm Double Flange, 1-2 in Hex (VexPro):6
- [Mate]: Timing Pulley (HTD 5mm) - 18T 9mm Double Flange, 1-2 in Hex (VexPro):6 ↔ Hex Shaft Collar 1-2 in (7552K500):34
- Mate:1076: VersaPlanetary (Fixed):1 ↔ Hex Shaft Collar 1-2 in (7552K500):34
- Flush:29: Hex Shaft Collar 1-2 in (7552K500):32 ↔ Hex Shaft Collar 1-2 in (7552K500):34
- Mate:1077: VersaPlanetary (Fixed):1 ↔ Hex Shaft Collar 1-2 in (7552K500):34
- Mate:1078: Timing Pulley (HTD 5mm) - 18T 9mm Double Flange, 1-2 in Hex (VexPro):6 ↔ Hex Shaft Collar 1-2 in (7552K500):34
- Mate:1079: VersaPlanetary (Fixed):1 ↔ Timing Pulley (HTD 5mm) - 18T 9mm Double Flange, 1-2 in Hex (VexPro):6
- Mate:1080: VersaPlanetary (Fixed):1 ↔ Timing Pulley (HTD 5mm) - 18T 9mm Double Flange, 1-2 in Hex (VexPro):6
- Mate:1081: Hex Shaft Collar 1-2 in (7552K500):33 ↔ Timing Pulley (HTD 5mm) - 18T 9mm Double Flange, 1-2 in Hex (VexPro):6
- Mate:1082: VersaPlanetary (Fixed):1 ↔ Hex Shaft Collar 1-2 in (7552K500):33
- Mate:1083: VersaPlanetary (Fixed):1 ↔ Hex Shaft Collar 1-2 in (7552K500):33
- Mate:1084: Vex Pro 1x1 rectangular tubing 14 in length:5 ↔ Vex Pro 90 degree gusset (1-8 in):3
- Mate:1085: Vex Pro 1x1 rectangular tubing 14 in length:5 ↔ Vex Pro 90 degree gusset (1-8 in):3
- Mate:1086: Vex Pro 1x1 rectangular tubing 2 in length:2 ↔ Vex Pro 90 degree gusset (1-8 in):3
- Mate:1090: Vex Pro 1x1 rectangular tubing 2 in length:4 ↔ Vex Pro 90 degree gusset (1-8 in):4
- Mate:1091: Vex Pro 1x1 rectangular tubing 2 in length:4 ↔ Vex Pro 90 degree gusset (1-8 in):4
- Mate:1092: Vex Pro 1x1 rectangular tubing 14 in length:6 ↔ Vex Pro 90 degree gusset (1-8 in):4
- Mate:1108: Roller End Cap Drive (3-D Printed):5 ↔ Hex Shaft Aluminum 1-2 in (am-2291):2
- Mate:1109: Roller End Cap Drive (3-D Printed):5 ↔ Hex Shaft Aluminum 1-2 in (am-2291):2
- Mate:1110: Roller End Cap Drive (3-D Printed):5 ↔ Hex Shaft Collar 1-2 in (7552K500):23
- Mate:1111: Hex Bearing 1-2 in (FR8ZZ-Hex, am-0279):6 ↔ Hex Shaft Collar 1-2 in (7552K500):23
- Mate:1112: Roller End Cap Drive (3-D Printed):2 ↔ Hex Shaft Collar 1-2 in (7552K500):22
- Mate:1113: Hex Bearing 1-2 in (FR8ZZ-Hex, am-0279):3 ↔ Hex Shaft Collar 1-2 in (7552K500):22
- Flush:30: Roller End Cap Drive (3-D Printed):2 ↔ Hex Shaft Aluminum 1-2 in (am-2291):1
- Mate:1114: Roller End Cap Drive (3-D Printed):2 ↔ Polycarbonate Roller 2 OD 1-16 Thick (8585K64):1
- Mate:1115: Roller End Cap Drive (3-D Printed):2 ↔ Polycarbonate Roller 2 OD 1-16 Thick (8585K64):1
- Mate:1117: Vex Pro 1x1 rectangular tubing 14 in length:6 ↔ Lexan flexible Arm Mount:1
- Mate:1123: Lexan flexible Arm Mount:2 ↔ Hex Shaft Connector (Lexan):1
- Mate:1124: Lexan flexible Arm Mount:2 ↔ Hex Shaft Connector (Lexan):1
- Mate:1125: Lexan flexible Arm Mount:2 ↔ Hex Shaft Connector (Lexan):1
- Mate:1126: Lexan flexible Arm Mount:1 ↔ Hex Shaft Connector (Lexan):2
- Mate:1127: Lexan flexible Arm Mount:1 ↔ Hex Shaft Connector (Lexan):2
- Mate:1128: Lexan flexible Arm Mount:1 ↔ Hex Shaft Connector (Lexan):2
- Mate:1129: Vex Pro 1x1 rectangular tubing 14 in length:6 ↔ Lexan flexible Arm Mount:1
- Mate:1130: Vex Pro 1x1 rectangular tubing 14 in length:6 ↔ Lexan flexible Arm Mount:1
- Mate:1131: Vex Pro 1x1 rectangular tubing 14 in length:6 ↔ Lexan flexible Arm Mount:2
- Mate:1132: Vex Pro 1x1 rectangular tubing 14 in length:6 ↔ Lexan flexible Arm Mount:2
- Mate:1133: Hex Shaft 1-2 in 5 in long (am-0856):1 ↔ Hex Shaft Connector (Lexan):1
- Mate:1134: Hex Shaft Collar 1-2 in (7552K500):30 ↔ Hex Shaft Connector (Lexan):1
- Mate:1135: Hex Shaft 1-2 in 5 in long (am-0856):1 ↔ Hex Shaft Connector (Lexan):2
- Mate:1136: Hex Shaft Collar 1-2 in (7552K500):21 ↔ Hex Shaft Connector (Lexan):2
- [Mate]: Lexan flexible Arm Mount:3 ↔ Hex Shaft Connector (Lexan):3
- [Mate]: Lexan flexible Arm Mount:3 ↔ Hex Shaft Connector (Lexan):3
- [Mate]: Lexan flexible Arm Mount:3 ↔ Hex Shaft Connector (Lexan):3
- Mate:1140: Vex Pro 1x1 rectangular tubing 14 in length:5 ↔ Lexan flexible Arm Mount:3
- Mate:1141: Vex Pro 1x1 rectangular tubing 14 in length:5 ↔ Lexan flexible Arm Mount:3
- [Mate]: Lexan flexible Arm Mount:4 ↔ Hex Shaft Connector (Lexan):4
- [Mate]: Lexan flexible Arm Mount:4 ↔ Hex Shaft Connector (Lexan):4
- [Mate]: Lexan flexible Arm Mount:4 ↔ Hex Shaft Connector (Lexan):4
- Mate:1146: Vex Pro 1x1 rectangular tubing 14 in length:5 ↔ Lexan flexible Arm Mount:4
- Mate:1147: Vex Pro 1x1 rectangular tubing 14 in length:5 ↔ Lexan flexible Arm Mount:4
- Mate:1148: Vex Pro 1x1 rectangular tubing 14 in length:5 ↔ Lexan flexible Arm Mount:4
- Mate:1149: Hex Shaft Collar 1-2 in (7552K500):19 ↔ Hex Shaft Connector (Lexan):4
- Mate:1150: Hex Shaft Collar 1-2 in (7552K500):18 ↔ Hex Shaft Connector (Lexan):3
- Mate:1153 (38.1 mm): Lexan flexible Arm Mount:1 ↔ Lexan flexible Arm Mount:2
- Mate:1154 (38.1 mm): Lexan flexible Arm Mount:3 ↔ Lexan flexible Arm Mount:4
- Mate:1155: Pneumatic Piston Front Flange (Rt Custom):2 ↔ Clamp with Piston Assembly (new):1
- Mate:1156: Pneumatic Piston Front Flange (Rt Custom):2 ↔ Clamp with Piston Assembly (new):1
- Mate:1157: Pneumatic Piston Front Flange (Rt Custom):2 ↔ Clamp with Piston Assembly (new):1
- Mate:1159: Hex Shaft Collar 3-8 in (7552K300):4 ↔ Clamp with Piston Assembly (new):1
- Mate:1160: Pneumatic Piston Front Flange (Lt Custom):1 ↔ Clamp with Piston Assembly (new):2
- Mate:1161: Pneumatic Piston Front Flange (Lt Custom):1 ↔ Clamp with Piston Assembly (new):2
- Mate:1162: Pneumatic Piston Front Flange (Lt Custom):1 ↔ Clamp with Piston Assembly (new):2
- Mate:1163: Hex Shaft Collar 3-8 in (7552K300):1 ↔ Clamp with Piston Assembly (new):2
- Mate:1164: Hex Shaft Collar 3-8 in (7552K300):2 ↔ Clamp with Piston Assembly (new):2
- Flush:32: Hex Shaft 3-8 in (am-0855):1 ↔ Hex Shaft Collar 3-8 in (7552K300):2
- Flush:33 (-15.875 mm): Hex Shaft 3-8 in (am-0855):1 ↔ Hex Spacer:7
- Mate:1166: Hex Shaft Collar 3-8 in (7552K300):7 ↔ Clamp with Piston Assembly (new):2
- Mate:1167: Hex Shaft Collar 3-8 in (7552K300):1 ↔ Clamp with Piston Assembly (new):2
- Flush:34: Hex Shaft 3-8 in (am-0855):2 ↔ Hex Shaft Collar 3-8 in (7552K300):4
- Mate:1168: Hex Shaft Collar 3-8 in (7552K300):8 ↔ Clamp with Piston Assembly (new):1
- Mate:1170: Hex Shaft Collar 3-8 in (7552K300):3 ↔ Clamp with Piston Assembly (new):1
- Mate:1183: Hex Shaft Collar 3-8 in (7552K300):3 ↔ Clamp with Piston Assembly (new):1
- Mate:1184: Vex Pro 1x1 rectangular tubing 14 in length:5 ↔ Vex Pro T gusset - OUT OF STOCK 1192014:1
- Mate:1185: Vex Pro 1x1 rectangular tubing 14 in length:5 ↔ Vex Pro T gusset - OUT OF STOCK 1192014:1
- Mate:1186: Vex Pro 1x1 rectangular tubing 14 in length:5 ↔ Vex Pro T gusset - OUT OF STOCK 1192014:1
- Mate:1187: Vex Pro 1x1 rectangular tubing 4 in length:3 ↔ Vex Pro T gusset - OUT OF STOCK 1192014:1
- Flush:35: Vex Pro 1x1 rectangular tubing 4 in length:3 ↔ Vex Pro T gusset - OUT OF STOCK 1192014:1
- Mate:1188: Vex Pro T gusset - OUT OF STOCK 1192014:1 ↔ Vex Pro 1x1 rectangular tubing 2 in length (no hex):1
- Mate:1189: Vex Pro T gusset - OUT OF STOCK 1192014:1 ↔ Vex Pro 1x1 rectangular tubing 2 in length (no hex):1
- Flush:36: Vex Pro T gusset - OUT OF STOCK 1192014:1 ↔ Vex Pro 1x1 rectangular tubing 2 in length (no hex):1
- Mate:1190: Vex Pro 1x1 rectangular tubing 14 in length:5 ↔ Vex Pro T gusset - OUT OF STOCK 1192014:2
- Mate:1191: Vex Pro 1x1 rectangular tubing 14 in length:5 ↔ Vex Pro T gusset - OUT OF STOCK 1192014:2
- Mate:1192: Vex Pro 1x1 rectangular tubing 14 in length:5 ↔ Vex Pro T gusset - OUT OF STOCK 1192014:2
- Mate:1193: Vex Pro 1x1 rectangular tubing 2 in length (no hex):1 ↔ Vex Pro T gusset - OUT OF STOCK 1192014:2
- Mate:1194: Vex Pro 1x1 rectangular tubing 4 in length:3 ↔ Vex Pro T gusset - OUT OF STOCK 1192014:2
- Mate:1195: Vex Pro 1x1 rectangular tubing 14 in length (roller):1 ↔ Roller Crossbar Gusset (Custom):5
- Mate:1196: Vex Pro 1x1 rectangular tubing 14 in length (roller):1 ↔ Roller Crossbar Gusset (Custom):5
- Mate:1197: Vex Pro 1x1 rectangular tubing 14 in length (roller):2 ↔ Roller Crossbar Gusset (Custom):4
- Mate:1198: Vex Pro 1x1 rectangular tubing 14 in length (roller):2 ↔ Roller Crossbar Gusset (Custom):4
- Mate:1199: Vex Pro 1x1 rectangular tubing 21.375 in length:1 ↔ Roller Crossbar Gusset (Custom):4
- Mate:1203: Clamp with Piston Assembly (new):2 ↔ Torsion Spring 10 in-lb (9271K621):1
- Flush:37 (-4.7625 mm): Vex Pro 1x1 rectangular tubing 2 in length:1 ↔ Torsion Spring 10 in-lb (9271K621):1
- Mate:1204: Clamp with Piston Assembly (new):2 ↔ Torsion Spring 10 in-lb (9271K621):2
- Flush:38 (-4.7625 mm): Vex Pro 1x1 rectangular tubing 2 in length:2 ↔ Torsion Spring 10 in-lb (9271K621):2
- Mate:1205: Hex Shaft Collar 3-8 in (7552K300):6 ↔ Clamp with Piston Assembly (new):2
- Mate:1206: Hex Shaft Collar 3-8 in (7552K300):5 ↔ Clamp with Piston Assembly (new):1
- Mate:1207: Clamp with Piston Assembly (new):1 ↔ Torsion Spring 10 in-lb (9271K621):3
- Mate:1208: Clamp with Piston Assembly (new):1 ↔ Torsion Spring 10 in-lb (9271K621):4
- Flush:40 (-4.7625 mm): Vex Pro 1x1 rectangular tubing 2 in length:3 ↔ Torsion Spring 10 in-lb (9271K621):4
- Mate:1211: Vex Pro 1x1 rectangular tubing 14 in length (roller):2 ↔ Roller Crossbar Gusset (Custom):6
- Mate:1212: Vex Pro 1x1 rectangular tubing 14 in length (roller):2 ↔ Roller Crossbar Gusset (Custom):6
- Mate:1213: Vex Pro 1x1 rectangular tubing 21.375 in length:1 ↔ Roller Crossbar Gusset (Custom):6
- Mate:1214: Vex Pro 1x1 rectangular tubing 14 in length (roller):1 ↔ Roller Crossbar Gusset (Custom):7
- Mate:1215: Vex Pro 1x1 rectangular tubing 14 in length (roller):1 ↔ Roller Crossbar Gusset (Custom):7
- Mate:1216: Vex Pro 1x1 rectangular tubing 14 in length (roller):1 ↔ Roller Crossbar Gusset (Custom):7
- Mate:1218: Vex Pro 1x1 rectangular tubing 14 in length:5 ↔ Bearing Mount Spacer 1-8 in:1
- Mate:1219: Vex Pro 1x1 rectangular tubing 14 in length:5 ↔ Bearing Mount Spacer 1-8 in:1
- Mate:1220: Vex Pro 1x1 rectangular tubing 14 in length:5 ↔ Bearing Mount Spacer 1-8 in:1
- Mate:1221: Vex Pro End Bearing Mount (Bolt):1 ↔ Bearing Mount Spacer 1-8 in:1
- Mate:1222: Vex Pro End Bearing Mount (Bolt):1 ↔ Bearing Mount Spacer 1-8 in:1